# Autodesk Inventor assembly: 部件1
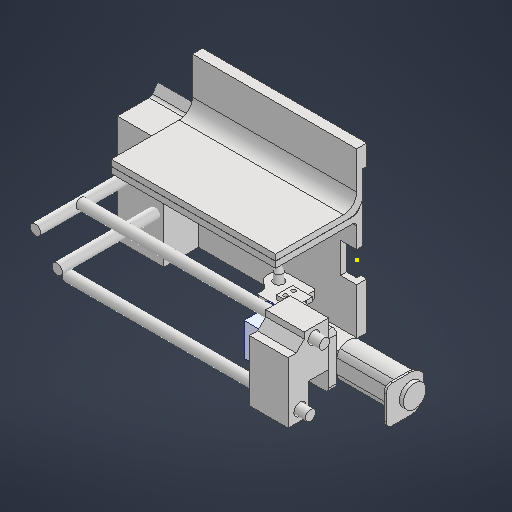
[picture p0: Inventor's stored thumbnail of the model, 512x512]
Saved by Autodesk Inventor 2025 (Build 290162000, 162)
## iProperties
Created: 2025-11-30
Part Number: 部件1
Document SubType Name: Assembly
Designer: XH
Author: XH
## Documents named in this file (8)
- D:\2 B Mechanical design\braille-printer-v2\部件1.iam
- D:\2 B Mechanical design\braille-printer-v2\便签.ipt
- D:\2 B Mechanical design\braille-printer-v2\主体.ipt
- D:\2 B Mechanical design\braille-printer-v2\前舵机位置控制.ipt
- D:\2 B Mechanical design\braille-printer-v2\针头主体.iam
- D:\2 B Mechanical design\braille-printer-v2\电机.ipt
- D:\2 B Mechanical design\braille-printer-v2\钢轴.ipt
- D:\2 B Mechanical design\braille-printer-v2\Y轴杠轴.ipt
## Components (9 placed, 7 different names)
1. 便签:1 — 配合:1, 配合:2, 配合:3
2. 主体:1 — 配合:1, 配合:2, 表面齐平:1, 表面齐平:4
3. 前舵机位置控制:1 — 配合:3, 表面齐平:1
4. 针头主体:1 [sub-assembly] — 配合:4, 配合:5
5. 电机:1
6. 钢轴:1 — 表面齐平:3, 配合:4
7. 钢轴:2 — 表面齐平:3, 配合:5, 表面齐平:4
8. Y轴杠轴:1 — 表面齐平:5
9. Y轴杠轴:2 — 表面齐平:5
## Relationships (9: Mate 5, Flush 4)
- 配合:1 [Mate]: 便签:1 ↔ 主体:1
- 配合:2 [Mate]: 便签:1 ↔ 主体:1
- 配合:3 [Mate]: 便签:1 ↔ 前舵机位置控制:1
- 表面齐平:1 [Flush]: 主体:1 ↔ 前舵机位置控制:1
- 表面齐平:3 [Flush]: 钢轴:1 ↔ 钢轴:2
- 配合:4 [Mate]: 针头主体:1 ↔ 钢轴:1
- 配合:5 [Mate]: 针头主体:1 ↔ 钢轴:2
- 表面齐平:4 [Flush] (5 mm): 主体:1 ↔ 钢轴:2
- 表面齐平:5 [Flush]: Y轴杠轴:1 ↔ Y轴杠轴:2
